# Autodesk Inventor assembly: wheel2_MIR
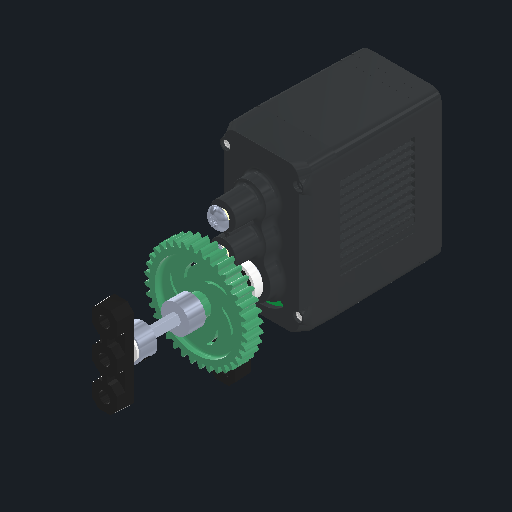
[picture p0: Inventor's stored thumbnail of the model, 512x512]
Saved by Autodesk Inventor 2024 (Build 280153000, 153)
## iProperties
Created: 2023-08-09
Part Number: wheel2_MIR
Document SubType Name: Assembly
Designer: macbook
Author: macbook
## Documents named in this file (11)
- \\Mac\Home\Desktop\code\7899V-VRC-OVER-UNDER\Cad\VEX-CAD-Inventor-1.4.0\Assembly\v0.2\wheel2_MIR.iam
- \\Mac\Home\Desktop\code\7899V-VRC-OVER-UNDER\Cad\VEX-CAD-Inventor-1.4.0\Motion\Gears\LS 36T Gear_MIR1.ipt
- \\Mac\Home\Desktop\code\7899V-VRC-OVER-UNDER\Cad\VEX-CAD-Inventor-1.4.0\Motion\Shaft LS\Bearing Flat_MIR1.ipt
- \\Mac\Home\Desktop\code\7899V-VRC-OVER-UNDER\Cad\VEX-CAD-Inventor-1.4.0\Motion\Shaft LS\Shaft LS\Shaft LS 2.5.ipt
- \\Mac\Home\Desktop\code\7899V-VRC-OVER-UNDER\Cad\VEX-CAD-Inventor-1.4.0\Motion\Shaft LS\Shaft LS.ipt
- \\Mac\Home\Desktop\code\7899V-VRC-OVER-UNDER\Cad\VEX-CAD-Inventor-1.4.0\Motion\Shaft LS\Shaft Collar Metal\Shaft Collar Set Screw_MIR.iam
- \\Mac\Home\Desktop\code\7899V-VRC-OVER-UNDER\Cad\VEX-CAD-Inventor-1.4.0\Electronics\Motors with Screws\AluM-StarS_MIR1.iam
- \\Mac\Home\Desktop\code\7899V-VRC-OVER-UNDER\Cad\VEX-CAD-Inventor-1.4.0\Motion\Spacers\Washer Teflon\TWasher .375 OD x .03125.ipt
- \\Mac\Home\Desktop\code\7899V-VRC-OVER-UNDER\Cad\VEX-CAD-Inventor-1.4.0\Motion\Spacers\Washer Teflon.ipt
- \\Mac\Home\Desktop\code\7899V-VRC-OVER-UNDER\Cad\VEX-CAD-Inventor-1.4.0\Motion\Spacers\Spacer Nylon .500 OD\NSpacer White .500 OD x .125.ipt
- \\Mac\Home\Desktop\code\7899V-VRC-OVER-UNDER\Cad\VEX-CAD-Inventor-1.4.0\Motion\Spacers\Spacer Nylon .500 OD.ipt
## Components (11 placed, 7 different names)
1. LS 36T Gear_MIR1:1 — Insert:2, Insert:1
2. Bearing Flat_MIR1:1 — Insert:16, Insert:14, Insert:12, Insert:18, Cylindrical:3
3. Shaft LS 2.5:1 — Mate:1, Cylindrical:3, Cylindrical:2
4. Shaft Collar Set Screw_MIR:1 [sub-assembly] — Insert:11
5. Shaft Collar Set Screw_MIR:2 [sub-assembly] — Insert:2, Cylindrical:2
6. AluM-StarS_MIR1:1 [sub-assembly] — Mate:1, Insert:15, Insert:13
7. TWasher .375 OD x .03125:1 — Insert:1, Insert:17
8. Bearing Flat_MIR1:2 — Insert:16, Insert:15, Insert:14, Insert:13
9. TWasher .375 OD x .03125:2 — Insert:12, Insert:11
10. Bearing Flat_MIR1:3 — Insert:18, Insert:17, Insert:19
11. NSpacer White .500 OD x .125:1 — Insert:19
## Relationships (14: Insert 11, CylindricalJoint 2, Mate 1)
- Insert:2: LS 36T Gear_MIR1:1 ↔ Shaft Collar Set Screw_MIR:2
- Mate:1: Shaft LS 2.5:1 ↔ AluM-StarS_MIR1:1
- Insert:1: LS 36T Gear_MIR1:1 ↔ TWasher .375 OD x .03125:1
- Insert:16: Bearing Flat_MIR1:1 ↔ Bearing Flat_MIR1:2
- Insert:15 (46.0375 mm): AluM-StarS_MIR1:1 ↔ Bearing Flat_MIR1:2
- Insert:14: Bearing Flat_MIR1:1 ↔ Bearing Flat_MIR1:2
- Insert:13 (46.0375 mm): AluM-StarS_MIR1:1 ↔ Bearing Flat_MIR1:2
- Insert:12 (1.5875 mm): Bearing Flat_MIR1:1 ↔ TWasher .375 OD x .03125:2
- Insert:11: Shaft Collar Set Screw_MIR:1 ↔ TWasher .375 OD x .03125:2
- Insert:18 (39.37 mm): Bearing Flat_MIR1:1 ↔ Bearing Flat_MIR1:3
- Insert:17 (1.5875 mm): TWasher .375 OD x .03125:1 ↔ Bearing Flat_MIR1:3
- Insert:19: Bearing Flat_MIR1:3 ↔ NSpacer White .500 OD x .125:1
- Cylindrical:3: Bearing Flat_MIR1:1 ↔ Shaft LS 2.5:1
- Cylindrical:2: Shaft LS 2.5:1 ↔ Shaft Collar Set Screw_MIR:2
